# Autodesk Inventor assembly: endAssembly
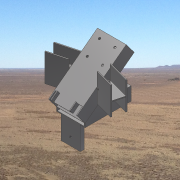
[picture p0: Inventor's stored thumbnail of the model, 180x180]
Saved by Autodesk Inventor 2014 SP1 (Build 180222100, 222)
## iProperties
Created: 2013-12-03
Part Number: endAssembly
Document SubType Name: Assembly
Designer: Dave
Author: Dave
## Documents named in this file (5)
- C:\Users\Dave\Desktop\hera-cad\support\endAssembly.iam
- C:\Users\Dave\Desktop\hera-cad\support\endHoriz.ipt
- C:\Users\Dave\Desktop\hera-cad\support\end37.ipt
- C:\Users\Dave\Desktop\hera-cad\support\endVert1.ipt
- C:\Users\Dave\Desktop\hera-cad\support\endVert1_MIR1.ipt
## Components (4 placed, 4 different names)
1. endHoriz:1 — Mate:1, Flush:3, Flush:4, Flush:6
2. end37:1 — Mate:1, Flush:3, Mate:7, Flush:5
3. endVert1:1 — Mate:7, Flush:4, Flush:6
4. endVert1_MIR1:1
## Relationships (6: Flush 4, Mate 2)
- Mate:1: endHoriz:1 ↔ end37:1
- Flush:3: endHoriz:1 ↔ end37:1
- Mate:7: end37:1 ↔ endVert1:1
- Flush:4 (-50.8 mm): endHoriz:1 ↔ endVert1:1
- Flush:5 (44.45 mm): end37:1
- Flush:6 (38.1 mm): endHoriz:1 ↔ endVert1:1
